# Autodesk Inventor assembly: McCrea_WALLE_bez_HEAD_walle
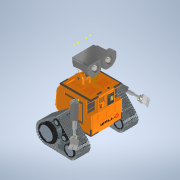
[picture p0: Inventor's stored thumbnail of the model, 180x180]
Saved by Autodesk Inventor 2022 (Build 260153000, 153)
## iProperties
Created: 2022-02-01
Part Number: McCrea_WALLE_bez_HEAD_walle
Document SubType Name: Assembly
Designer: MatusBarany
Author: MatusBarany
## Documents named in this file (5)
- C:\Users\Lukas\Desktop\ard\3D\Walle\FINAL\assembly\McCrea_WALLE_bez_HEAD_walle.iam
- C:\Users\Lukas\Desktop\ard\3D\Walle\FINAL\lukas\McCrea_RUKA_TELO_SPOJ_walle.iam
- C:\Users\Lukas\Desktop\ard\3D\Walle\FINAL\matus\McCrea_pasy_zlozene_walle.iam
- C:\Users\Lukas\Desktop\ard\3D\Walle\FINAL\matus\McCrea_pasy_zlozene_walle_MIR.iam
- C:\Users\Lukas\Desktop\ard\3D\Walle\FINAL\assembly\McCrea_head_walle.iam
## Components (4 placed, 4 different names)
1. McCrea_RUKA_TELO_SPOJ_walle:1 [sub-assembly] — Mate:1, Mate:2, Mate:3, Mate:4, Mate:5, Mate:6, Mate:7, Mate:8, Mate:9
2. McCrea_pasy_zlozene_walle:1 [sub-assembly] — Mate:1, Mate:2, Mate:3
3. McCrea_pasy_zlozene_walle_MIR:1 [sub-assembly] — Mate:7, Mate:8, Mate:9
4. McCrea_head_walle:1 [sub-assembly] — Mate:4, Mate:5, Mate:6
## Relationships (9: Mate 9)
- Mate:1: McCrea_RUKA_TELO_SPOJ_walle:1 ↔ McCrea_pasy_zlozene_walle:1
- Mate:2: McCrea_RUKA_TELO_SPOJ_walle:1 ↔ McCrea_pasy_zlozene_walle:1
- Mate:3: McCrea_RUKA_TELO_SPOJ_walle:1 ↔ McCrea_pasy_zlozene_walle:1
- Mate:4: McCrea_RUKA_TELO_SPOJ_walle:1 ↔ McCrea_head_walle:1
- Mate:5: McCrea_RUKA_TELO_SPOJ_walle:1 ↔ McCrea_head_walle:1
- Mate:6: McCrea_RUKA_TELO_SPOJ_walle:1 ↔ McCrea_head_walle:1
- Mate:7: McCrea_RUKA_TELO_SPOJ_walle:1 ↔ McCrea_pasy_zlozene_walle_MIR:1
- Mate:8: McCrea_RUKA_TELO_SPOJ_walle:1 ↔ McCrea_pasy_zlozene_walle_MIR:1
- Mate:9: McCrea_RUKA_TELO_SPOJ_walle:1 ↔ McCrea_pasy_zlozene_walle_MIR:1
